# Autodesk Inventor assembly: Camera-Unit Back
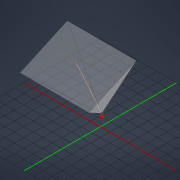
[picture p0: Inventor's stored thumbnail of the model, 180x180]
Saved by Autodesk Inventor 2022.2 (Build 262287010, 287A)
## iProperties
Created: 2022-04-02
Part Number: Camera-Unit Back
Document SubType Name: Assembly
Designer: sleib
Author: sleib
## Documents named in this file (6)
- C:\Users\sleib\Projekte\Voron-2\CAD\Inventor\Camera-Unit Back.iam
- C:\Users\sleib\Projekte\Voron-2\CAD\Inventor\Camera-Mount.ipt
- C:\Users\sleib\Projekte\Voron-2\CAD\Inventor\M3 Threaded Insert.ipt
- C:\Users\sleib\Projekte\Voron-2\CAD\Inventor\Camera-Base.ipt
- C:\Users\sleib\Projekte\Voron-2\CAD\Inventor\Cam V2.1 v1.ipt
- C:\Users\sleib\Projekte\Voron-2\CAD\Inventor\Camera-Viewcone.ipt
## Components (6 placed, 5 different names)
1. Camera-Mount:1 — Passend:1, Passend:2, Fluchtend:1, Fluchtend:2, Passend:5
2. M3 Threaded Insert:1 — Passend:1, Fluchtend:1, Passend:4
3. M3 Threaded Insert:2 — Passend:2, Fluchtend:2, Passend:3
4. Camera-Base:1 — Passend:3, Passend:4, Passend:5, Passend:6, Passend:7, Passend:8, Passend:9, Passend:10
5. Cam V2.1 v1:1 — Passend:6, Passend:7, Passend:8, Passend:9, Passend:10, Passend:11, Winkel:1, Fluchtend:3, Passend:12
6. Camera-Viewcone:1 — Passend:11, Winkel:1, Fluchtend:3, Passend:12
## Relationships (16: Mate 12, Flush 3, Angle 1)
- Passend:1 [Mate]: Camera-Mount:1 ↔ M3 Threaded Insert:1
- Passend:2 [Mate]: Camera-Mount:1 ↔ M3 Threaded Insert:2
- Fluchtend:1 [Flush]: Camera-Mount:1 ↔ M3 Threaded Insert:1
- Fluchtend:2 [Flush]: Camera-Mount:1 ↔ M3 Threaded Insert:2
- Passend:3 [Mate]: M3 Threaded Insert:2 ↔ Camera-Base:1
- Passend:4 [Mate]: M3 Threaded Insert:1 ↔ Camera-Base:1
- Passend:5 [Mate]: Camera-Mount:1 ↔ Camera-Base:1
- Passend:6 [Mate]: Camera-Base:1 ↔ Cam V2.1 v1:1
- Passend:7 [Mate]: Camera-Base:1 ↔ Cam V2.1 v1:1
- Passend:8 [Mate]: Camera-Base:1 ↔ Cam V2.1 v1:1
- Passend:9 [Mate]: Camera-Base:1 ↔ Cam V2.1 v1:1
- Passend:10 [Mate] (7 mm): Camera-Base:1 ↔ Cam V2.1 v1:1
- Passend:11 [Mate]: Cam V2.1 v1:1 ↔ Camera-Viewcone:1
- Winkel:1 [Angle] (0 deg): Cam V2.1 v1:1 ↔ Camera-Viewcone:1
- Fluchtend:3 [Flush]: Cam V2.1 v1:1 ↔ Camera-Viewcone:1
- Passend:12 [Mate]: Cam V2.1 v1:1 ↔ Camera-Viewcone:1
